# Autodesk Inventor assembly: Shin Impact V1.0
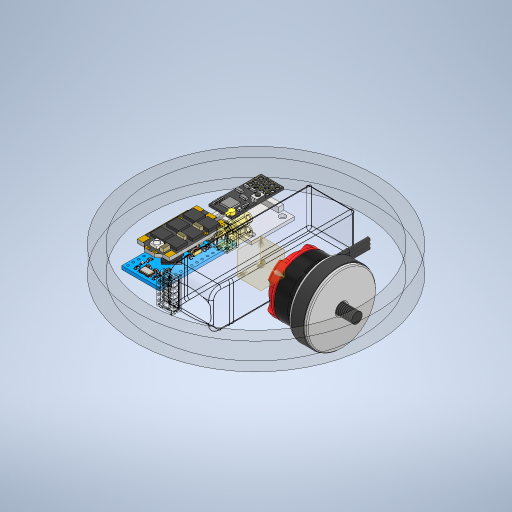
[picture p0: Inventor's stored thumbnail of the model, 512x512]
Saved by Autodesk Inventor 2023.4 (Build 274418000, 418)
## iProperties
Created: 2023-01-05
Part Number: Shin Impact V1.0
Document SubType Name: Assembly
Designer: Nathan Cai
Mass: 308.512 g
Surface Area: 482.426 cm^2
Volume: 44.9162 cm^3
Density: 6.86861 g/cm^3
Author: Nathan Cai
## Documents named in this file (10)
- E:\Documents\Inventor\Shin Impact V1.0\Shin Impact V1.0.iam
- E:\Documents\Inventor\Shin Impact V1.0\ProMicro\ProMicro.iam
- E:\Documents\Inventor\Shin Impact V1.0\H3LIS331DL.ipt
- E:\Documents\Inventor\Shin Impact V1.0\AKK RS2205 2300KV\AKK RS2205 2300KV.iam
- E:\Documents\Inventor\Shin Impact V1.0\GT2 Pulley Generator.ipt
- E:\Documents\Inventor\Shin Impact V1.0\GT2 Belt Generator.ipt
- E:\Documents\Inventor\Shin Impact V1.0\Tattu 3S 550mah\Tattu 550mah 3S.iam
- E:\Documents\Inventor\Shin Impact V1.0\RDQ ESC32.ipt
- E:\Documents\Inventor\Shin Impact V1.0\Receptor FS2A mini\Receptor FS2A mini.ipt
- E:\Documents\Inventor\Shin Impact V1.0\Blade.ipt
## Components (9 placed, 9 different names)
1. ProMicro:1 [sub-assembly]
2. H3LIS331DL:1
3. AKK RS2205 2300KV:1 [sub-assembly] — Mate:1, Mate:2
4. GT2 Pulley Generator:1 — Mate:1, Mate:2, Mate:3, Mate:4, Mate:5
5. GT2 Belt Generator:1 — Mate:3, Mate:4, Mate:5
6. Tattu 550mah 3S:1 [sub-assembly]
7. RDQ ESC32:1
8. Receptor FS2A mini:1
9. Blade:1
## Relationships (5: Mate 5)
- Mate:1: AKK RS2205 2300KV:1 ↔ GT2 Pulley Generator:1
- Mate:2 (-2 mm): AKK RS2205 2300KV:1 ↔ GT2 Pulley Generator:1
- Mate:3: GT2 Pulley Generator:1 ↔ GT2 Belt Generator:1
- Mate:4: GT2 Pulley Generator:1 ↔ GT2 Belt Generator:1
- Mate:5: GT2 Pulley Generator:1 ↔ GT2 Belt Generator:1
